# Autodesk Inventor assembly: Ambient_board_Meteostanice
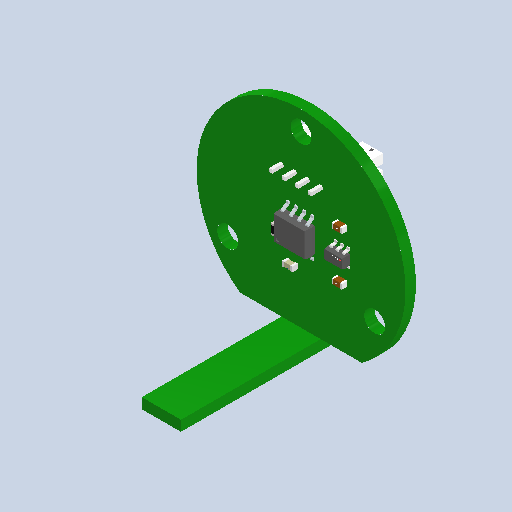
[picture p0: Inventor's stored thumbnail of the model, 512x512]
Saved by Autodesk Inventor 2025.2 (Build 292293000, 293)
## iProperties
Company: Open CASCADE
Created: 2025-02-10
Part Number: Ambient_board_Meteostanice
Description: Open CASCADE Model
Document SubType Name: Assembly
Designer: yehorderehus
Authority: Unknown
Sending System: Open CASCADE 7.5
Preprocessor: Open CASCADE STEP processor 7.5
Title: Open CASCADE Shape Model
Author: Author
## Documents named in this file (66)
- G:\.shortcut-targets-by-id\1Afqr12NmjXaFk11r_F7oLitoDl4TiMfc\Structures\assembly\Ambient_board_Meteostanice.iam
- G:\.shortcut-targets-by-id\1Afqr12NmjXaFk11r_F7oLitoDl4TiMfc\Structures\assembly\Ambient_board_Meteostanice\Ambient_board_Meteostanice\Open CASCADE STEP translator 7.5 66.ipt
- G:\.shortcut-targets-by-id\1Afqr12NmjXaFk11r_F7oLitoDl4TiMfc\Structures\assembly\Ambient_board_Meteostanice\Ambient_board_Meteostanice\Open CASCADE STEP translator 7.5 67.ipt
- G:\.shortcut-targets-by-id\1Afqr12NmjXaFk11r_F7oLitoDl4TiMfc\Structures\assembly\Ambient_board_Meteostanice\Ambient_board_Meteostanice\Open CASCADE STEP translator 7.5 68.ipt
- G:\.shortcut-targets-by-id\1Afqr12NmjXaFk11r_F7oLitoDl4TiMfc\Structures\assembly\Ambient_board_Meteostanice\Ambient_board_Meteostanice\Open CASCADE STEP translator 7.5 69.ipt
- G:\.shortcut-targets-by-id\1Afqr12NmjXaFk11r_F7oLitoDl4TiMfc\Structures\assembly\Ambient_board_Meteostanice\Ambient_board_Meteostanice\Open CASCADE STEP translator 7.5 70.ipt
- G:\.shortcut-targets-by-id\1Afqr12NmjXaFk11r_F7oLitoDl4TiMfc\Structures\assembly\Ambient_board_Meteostanice\Ambient_board_Meteostanice\Open CASCADE STEP translator 7.5 71.ipt
- G:\.shortcut-targets-by-id\1Afqr12NmjXaFk11r_F7oLitoDl4TiMfc\Structures\assembly\Ambient_board_Meteostanice\Ambient_board_Meteostanice\Open CASCADE STEP translator 7.5 72.ipt
- G:\.shortcut-targets-by-id\1Afqr12NmjXaFk11r_F7oLitoDl4TiMfc\Structures\assembly\Ambient_board_Meteostanice\Ambient_board_Meteostanice\Open CASCADE STEP translator 7.5 73.ipt
- G:\.shortcut-targets-by-id\1Afqr12NmjXaFk11r_F7oLitoDl4TiMfc\Structures\assembly\Ambient_board_Meteostanice\Ambient_board_Meteostanice\Open CASCADE STEP translator 7.5 74.ipt
- G:\.shortcut-targets-by-id\1Afqr12NmjXaFk11r_F7oLitoDl4TiMfc\Structures\assembly\Ambient_board_Meteostanice\Ambient_board_Meteostanice\Open CASCADE STEP translator 7.5 75.ipt
- G:\.shortcut-targets-by-id\1Afqr12NmjXaFk11r_F7oLitoDl4TiMfc\Structures\assembly\Ambient_board_Meteostanice\Ambient_board_Meteostanice\Open CASCADE STEP translator 7.5 76.ipt
- G:\.shortcut-targets-by-id\1Afqr12NmjXaFk11r_F7oLitoDl4TiMfc\Structures\assembly\Ambient_board_Meteostanice\Ambient_board_Meteostanice\Open CASCADE STEP translator 7.5 77.ipt
- G:\.shortcut-targets-by-id\1Afqr12NmjXaFk11r_F7oLitoDl4TiMfc\Structures\assembly\Ambient_board_Meteostanice\Ambient_board_Meteostanice\Open CASCADE STEP translator 7.5 78.ipt
- G:\.shortcut-targets-by-id\1Afqr12NmjXaFk11r_F7oLitoDl4TiMfc\Structures\assembly\Ambient_board_Meteostanice\Ambient_board_Meteostanice\Open CASCADE STEP translator 7.5 79.ipt
- G:\.shortcut-targets-by-id\1Afqr12NmjXaFk11r_F7oLitoDl4TiMfc\Structures\assembly\Ambient_board_Meteostanice\Ambient_board_Meteostanice\Open CASCADE STEP translator 7.5 80.ipt
- G:\.shortcut-targets-by-id\1Afqr12NmjXaFk11r_F7oLitoDl4TiMfc\Structures\assembly\Ambient_board_Meteostanice\Ambient_board_Meteostanice\Open CASCADE STEP translator 7.5 81.ipt
- G:\.shortcut-targets-by-id\1Afqr12NmjXaFk11r_F7oLitoDl4TiMfc\Structures\assembly\Ambient_board_Meteostanice\Ambient_board_Meteostanice\Open CASCADE STEP translator 7.5 82.ipt
- G:\.shortcut-targets-by-id\1Afqr12NmjXaFk11r_F7oLitoDl4TiMfc\Structures\assembly\Ambient_board_Meteostanice\Ambient_board_Meteostanice\Open CASCADE STEP translator 7.5 83.ipt
- G:\.shortcut-targets-by-id\1Afqr12NmjXaFk11r_F7oLitoDl4TiMfc\Structures\assembly\Ambient_board_Meteostanice\Ambient_board_Meteostanice\Open CASCADE STEP translator 7.5 84.ipt
- G:\.shortcut-targets-by-id\1Afqr12NmjXaFk11r_F7oLitoDl4TiMfc\Structures\assembly\Ambient_board_Meteostanice\Ambient_board_Meteostanice\Open CASCADE STEP translator 7.5 85.ipt
- G:\.shortcut-targets-by-id\1Afqr12NmjXaFk11r_F7oLitoDl4TiMfc\Structures\assembly\Ambient_board_Meteostanice\Ambient_board_Meteostanice\Open CASCADE STEP translator 7.5 86.ipt
- G:\.shortcut-targets-by-id\1Afqr12NmjXaFk11r_F7oLitoDl4TiMfc\Structures\assembly\Ambient_board_Meteostanice\Ambient_board_Meteostanice\Open CASCADE STEP translator 7.5 87.ipt
- G:\.shortcut-targets-by-id\1Afqr12NmjXaFk11r_F7oLitoDl4TiMfc\Structures\assembly\Ambient_board_Meteostanice\Ambient_board_Meteostanice\Open CASCADE STEP translator 7.5 88.ipt
- G:\.shortcut-targets-by-id\1Afqr12NmjXaFk11r_F7oLitoDl4TiMfc\Structures\assembly\Ambient_board_Meteostanice\Ambient_board_Meteostanice\Open CASCADE STEP translator 7.5 89.ipt
- G:\.shortcut-targets-by-id\1Afqr12NmjXaFk11r_F7oLitoDl4TiMfc\Structures\assembly\Ambient_board_Meteostanice\Ambient_board_Meteostanice\Open CASCADE STEP translator 7.5 90.ipt
- G:\.shortcut-targets-by-id\1Afqr12NmjXaFk11r_F7oLitoDl4TiMfc\Structures\assembly\Ambient_board_Meteostanice\Ambient_board_Meteostanice\Open CASCADE STEP translator 7.5 91.ipt
- G:\.shortcut-targets-by-id\1Afqr12NmjXaFk11r_F7oLitoDl4TiMfc\Structures\assembly\Ambient_board_Meteostanice\Ambient_board_Meteostanice\Open CASCADE STEP translator 7.5 92.ipt
- G:\.shortcut-targets-by-id\1Afqr12NmjXaFk11r_F7oLitoDl4TiMfc\Structures\assembly\Ambient_board_Meteostanice\Ambient_board_Meteostanice\Open CASCADE STEP translator 7.5 93.ipt
- G:\.shortcut-targets-by-id\1Afqr12NmjXaFk11r_F7oLitoDl4TiMfc\Structures\assembly\Ambient_board_Meteostanice\Ambient_board_Meteostanice\Open CASCADE STEP translator 7.5 94.ipt
- G:\.shortcut-targets-by-id\1Afqr12NmjXaFk11r_F7oLitoDl4TiMfc\Structures\assembly\Ambient_board_Meteostanice\Ambient_board_Meteostanice\Open CASCADE STEP translator 7.5 95.ipt
- G:\.shortcut-targets-by-id\1Afqr12NmjXaFk11r_F7oLitoDl4TiMfc\Structures\assembly\Ambient_board_Meteostanice\Ambient_board_Meteostanice\Open CASCADE STEP translator 7.5 96.ipt
- G:\.shortcut-targets-by-id\1Afqr12NmjXaFk11r_F7oLitoDl4TiMfc\Structures\assembly\Ambient_board_Meteostanice\Ambient_board_Meteostanice\Open CASCADE STEP translator 7.5 97.ipt
- G:\.shortcut-targets-by-id\1Afqr12NmjXaFk11r_F7oLitoDl4TiMfc\Structures\assembly\Ambient_board_Meteostanice\Ambient_board_Meteostanice\Open CASCADE STEP translator 7.5 101.ipt
- G:\.shortcut-targets-by-id\1Afqr12NmjXaFk11r_F7oLitoDl4TiMfc\Structures\assembly\Ambient_board_Meteostanice\Ambient_board_Meteostanice\Open CASCADE STEP translator 7.5 102.ipt
- G:\.shortcut-targets-by-id\1Afqr12NmjXaFk11r_F7oLitoDl4TiMfc\Structures\assembly\Ambient_board_Meteostanice\Ambient_board_Meteostanice\Open CASCADE STEP translator 7.5 103.ipt
- G:\.shortcut-targets-by-id\1Afqr12NmjXaFk11r_F7oLitoDl4TiMfc\Structures\assembly\Ambient_board_Meteostanice\Ambient_board_Meteostanice\Open CASCADE STEP translator 7.5 104.ipt
- G:\.shortcut-targets-by-id\1Afqr12NmjXaFk11r_F7oLitoDl4TiMfc\Structures\assembly\Ambient_board_Meteostanice\Ambient_board_Meteostanice\Open CASCADE STEP translator 7.5 105.ipt
- G:\.shortcut-targets-by-id\1Afqr12NmjXaFk11r_F7oLitoDl4TiMfc\Structures\assembly\Ambient_board_Meteostanice\Ambient_board_Meteostanice\Open CASCADE STEP translator 7.5 106.ipt
- G:\.shortcut-targets-by-id\1Afqr12NmjXaFk11r_F7oLitoDl4TiMfc\Structures\assembly\Ambient_board_Meteostanice\Ambient_board_Meteostanice\Open CASCADE STEP translator 7.5 107.ipt
- G:\.shortcut-targets-by-id\1Afqr12NmjXaFk11r_F7oLitoDl4TiMfc\Structures\assembly\Ambient_board_Meteostanice\Ambient_board_Meteostanice\Open CASCADE STEP translator 7.5 108.ipt
- G:\.shortcut-targets-by-id\1Afqr12NmjXaFk11r_F7oLitoDl4TiMfc\Structures\assembly\Ambient_board_Meteostanice\Ambient_board_Meteostanice\Open CASCADE STEP translator 7.5 109.ipt
- G:\.shortcut-targets-by-id\1Afqr12NmjXaFk11r_F7oLitoDl4TiMfc\Structures\assembly\Ambient_board_Meteostanice\Ambient_board_Meteostanice\Open CASCADE STEP translator 7.5 110.ipt
- G:\.shortcut-targets-by-id\1Afqr12NmjXaFk11r_F7oLitoDl4TiMfc\Structures\assembly\Ambient_board_Meteostanice\Ambient_board_Meteostanice\Open CASCADE STEP translator 7.5 111.ipt
- G:\.shortcut-targets-by-id\1Afqr12NmjXaFk11r_F7oLitoDl4TiMfc\Structures\assembly\Ambient_board_Meteostanice\Ambient_board_Meteostanice\Open CASCADE STEP translator 7.5 112.ipt
- G:\.shortcut-targets-by-id\1Afqr12NmjXaFk11r_F7oLitoDl4TiMfc\Structures\assembly\Ambient_board_Meteostanice\Ambient_board_Meteostanice\Open CASCADE STEP translator 7.5 113.ipt
- G:\.shortcut-targets-by-id\1Afqr12NmjXaFk11r_F7oLitoDl4TiMfc\Structures\assembly\Ambient_board_Meteostanice\Ambient_board_Meteostanice\Open CASCADE STEP translator 7.5 114.ipt
- G:\.shortcut-targets-by-id\1Afqr12NmjXaFk11r_F7oLitoDl4TiMfc\Structures\assembly\Ambient_board_Meteostanice\Ambient_board_Meteostanice\Open CASCADE STEP translator 7.5 115.ipt
- G:\.shortcut-targets-by-id\1Afqr12NmjXaFk11r_F7oLitoDl4TiMfc\Structures\assembly\Ambient_board_Meteostanice\Ambient_board_Meteostanice\Open CASCADE STEP translator 7.5 116.ipt
- G:\.shortcut-targets-by-id\1Afqr12NmjXaFk11r_F7oLitoDl4TiMfc\Structures\assembly\Ambient_board_Meteostanice\Ambient_board_Meteostanice\Open CASCADE STEP translator 7.5 117.ipt
- G:\.shortcut-targets-by-id\1Afqr12NmjXaFk11r_F7oLitoDl4TiMfc\Structures\assembly\Ambient_board_Meteostanice\Ambient_board_Meteostanice\Open CASCADE STEP translator 7.5 118.ipt
- G:\.shortcut-targets-by-id\1Afqr12NmjXaFk11r_F7oLitoDl4TiMfc\Structures\assembly\Ambient_board_Meteostanice\Ambient_board_Meteostanice\Open CASCADE STEP translator 7.5 119.ipt
- G:\.shortcut-targets-by-id\1Afqr12NmjXaFk11r_F7oLitoDl4TiMfc\Structures\assembly\Ambient_board_Meteostanice\Ambient_board_Meteostanice\Open CASCADE STEP translator 7.5 120.ipt
- G:\.shortcut-targets-by-id\1Afqr12NmjXaFk11r_F7oLitoDl4TiMfc\Structures\assembly\Ambient_board_Meteostanice\Ambient_board_Meteostanice\Open CASCADE STEP translator 7.5 121.ipt
- G:\.shortcut-targets-by-id\1Afqr12NmjXaFk11r_F7oLitoDl4TiMfc\Structures\assembly\Ambient_board_Meteostanice\Ambient_board_Meteostanice\Open CASCADE STEP translator 7.5 125.ipt
- G:\.shortcut-targets-by-id\1Afqr12NmjXaFk11r_F7oLitoDl4TiMfc\Structures\assembly\Ambient_board_Meteostanice\Ambient_board_Meteostanice\Open CASCADE STEP translator 7.5 126.ipt
- G:\.shortcut-targets-by-id\1Afqr12NmjXaFk11r_F7oLitoDl4TiMfc\Structures\assembly\Ambient_board_Meteostanice\Ambient_board_Meteostanice\Open CASCADE STEP translator 7.5 127.ipt
- G:\.shortcut-targets-by-id\1Afqr12NmjXaFk11r_F7oLitoDl4TiMfc\Structures\assembly\Ambient_board_Meteostanice\Ambient_board_Meteostanice\Open CASCADE STEP translator 7.5 128.ipt
- G:\.shortcut-targets-by-id\1Afqr12NmjXaFk11r_F7oLitoDl4TiMfc\Structures\assembly\Ambient_board_Meteostanice\Ambient_board_Meteostanice\Open CASCADE STEP translator 7.5 129.ipt
- G:\.shortcut-targets-by-id\1Afqr12NmjXaFk11r_F7oLitoDl4TiMfc\Structures\assembly\Ambient_board_Meteostanice\Ambient_board_Meteostanice\Open CASCADE STEP translator 7.5 130.ipt
- G:\.shortcut-targets-by-id\1Afqr12NmjXaFk11r_F7oLitoDl4TiMfc\Structures\assembly\Ambient_board_Meteostanice\Ambient_board_Meteostanice\Open CASCADE STEP translator 7.5 66_CPY1.ipt
- G:\.shortcut-targets-by-id\1Afqr12NmjXaFk11r_F7oLitoDl4TiMfc\Structures\assembly\Ambient_board_Meteostanice\Ambient_board_Meteostanice\Open CASCADE STEP translator 7.5 98_CPY.ipt
- G:\.shortcut-targets-by-id\1Afqr12NmjXaFk11r_F7oLitoDl4TiMfc\Structures\assembly\Ambient_board_Meteostanice\Ambient_board_Meteostanice\Open CASCADE STEP translator 7.5 99_CPY.ipt
- G:\.shortcut-targets-by-id\1Afqr12NmjXaFk11r_F7oLitoDl4TiMfc\Structures\assembly\Ambient_board_Meteostanice\Ambient_board_Meteostanice\Open CASCADE STEP translator 7.5 100_CPY.ipt
- G:\.shortcut-targets-by-id\1Afqr12NmjXaFk11r_F7oLitoDl4TiMfc\Structures\assembly\Ambient_board_Meteostanice\Ambient_board_Meteostanice\Open CASCADE STEP translator 7.5 123_CPY.ipt
- G:\.shortcut-targets-by-id\1Afqr12NmjXaFk11r_F7oLitoDl4TiMfc\Structures\assembly\Ambient_board_Meteostanice\Ambient_board_Meteostanice\Open CASCADE STEP translator 7.5 124_CPY.ipt
## Components (65 placed, 7 different names)
1. Open CASCADE STEP translator 7 — Rigid:1
2. Open CASCADE STEP translator 7:1
3. Open CASCADE STEP translator 7:2
4. Open CASCADE STEP translator 7:3
5. Open CASCADE STEP translator 7:4
6. Open CASCADE STEP translator 7:5
7. Open CASCADE STEP translator 7:6
8. Open CASCADE STEP translator 7:7
9. Open CASCADE STEP translator 7:8
10. Open CASCADE STEP translator 7:9
11. Open CASCADE STEP translator 7:10
12. Open CASCADE STEP translator 7:11
13. Open CASCADE STEP translator 7:12
14. Open CASCADE STEP translator 7:13
15. Open CASCADE STEP translator 7:14
16. Open CASCADE STEP translator 7:15
17. Open CASCADE STEP translator 7:16
18. Open CASCADE STEP translator 7:17
19. Open CASCADE STEP translator 7:18
20. Open CASCADE STEP translator 7:19
21. Open CASCADE STEP translator 7:20
22. Open CASCADE STEP translator 7:21
23. Open CASCADE STEP translator 7:22
24. Open CASCADE STEP translator 7:23
25. Open CASCADE STEP translator 7:24
26. Open CASCADE STEP translator 7:25
27. Open CASCADE STEP translator 7:26
28. Open CASCADE STEP translator 7:27
29. Open CASCADE STEP translator 7:28
30. Open CASCADE STEP translator 7:29
31. Open CASCADE STEP translator 7:30
32. Open CASCADE STEP translator 7:31
33. Open CASCADE STEP translator 7:35
34. Open CASCADE STEP translator 7:36
35. Open CASCADE STEP translator 7:37
36. Open CASCADE STEP translator 7:38
37. Open CASCADE STEP translator 7:39
38. Open CASCADE STEP translator 7:40
39. Open CASCADE STEP translator 7:41
40. Open CASCADE STEP translator 7:42
41. Open CASCADE STEP translator 7:43
42. Open CASCADE STEP translator 7:44
43. Open CASCADE STEP translator 7:45
44. Open CASCADE STEP translator 7:46
45. Open CASCADE STEP translator 7:47
46. Open CASCADE STEP translator 7:48
47. Open CASCADE STEP translator 7:49
48. Open CASCADE STEP translator 7:50
49. Open CASCADE STEP translator 7:51
50. Open CASCADE STEP translator 7:52
51. Open CASCADE STEP translator 7:53
52. Open CASCADE STEP translator 7:54
53. Open CASCADE STEP translator 7:55
54. Open CASCADE STEP translator 7:59
55. Open CASCADE STEP translator 7:60
56. Open CASCADE STEP translator 7:61
57. Open CASCADE STEP translator 7:62
58. Open CASCADE STEP translator 7:63
59. Open CASCADE STEP translator 7:64
60. Open CASCADE STEP translator 7.5 66_CPY1:1 — Flush:1, Flush:2, Flush:3, Flush:4, Flush:5, Flush:6, Flush:7, Flush:8, Flush:9, Flush:10, Flush:11, Flush:12, Flush:13, Mate:1, Flush:14, Rigid:1
61. Open CASCADE STEP translator 7.5 98_CPY:1 — Flush:3, Flush:8, Flush:13
62. Open CASCADE STEP translator 7.5 99_CPY:1 — Flush:5, Flush:10, Mate:1
63. Open CASCADE STEP translator 7.5 100_CPY:1 — Flush:4, Flush:9, Flush:14
64. Open CASCADE STEP translator 7.5 123_CPY:1 — Flush:1, Flush:7, Flush:11
65. Open CASCADE STEP translator 7.5 124_CPY:1 — Flush:2, Flush:6, Flush:12
## Relationships (16: Flush 14, Mate 1, WeldJoint 1)
- Flush:1 (-0.82 mm): Open CASCADE STEP translator 7.5 66_CPY1:1 ↔ Open CASCADE STEP translator 7.5 123_CPY:1
- Flush:2 (-0.87 mm): Open CASCADE STEP translator 7.5 66_CPY1:1 ↔ Open CASCADE STEP translator 7.5 124_CPY:1
- Flush:3 (-1.45 mm): Open CASCADE STEP translator 7.5 66_CPY1:1 ↔ Open CASCADE STEP translator 7.5 98_CPY:1
- Flush:4 (-0.766 mm): Open CASCADE STEP translator 7.5 66_CPY1:1 ↔ Open CASCADE STEP translator 7.5 100_CPY:1
- Flush:5 (-0.766 mm): Open CASCADE STEP translator 7.5 66_CPY1:1 ↔ Open CASCADE STEP translator 7.5 99_CPY:1
- Flush:6 (2.962 mm): Open CASCADE STEP translator 7.5 66_CPY1:1 ↔ Open CASCADE STEP translator 7.5 124_CPY:1
- Flush:7 (6.09 mm): Open CASCADE STEP translator 7.5 66_CPY1:1 ↔ Open CASCADE STEP translator 7.5 123_CPY:1
- Flush:8 (1.54 mm): Open CASCADE STEP translator 7.5 66_CPY1:1 ↔ Open CASCADE STEP translator 7.5 98_CPY:1
- Flush:9 (2.8 mm): Open CASCADE STEP translator 7.5 66_CPY1:1 ↔ Open CASCADE STEP translator 7.5 100_CPY:1
- Flush:10 (1.85 mm): Open CASCADE STEP translator 7.5 66_CPY1:1 ↔ Open CASCADE STEP translator 7.5 99_CPY:1
- Flush:11 (3.312 mm): Open CASCADE STEP translator 7.5 66_CPY1:1 ↔ Open CASCADE STEP translator 7.5 123_CPY:1
- Flush:12 (6.04 mm): Open CASCADE STEP translator 7.5 66_CPY1:1 ↔ Open CASCADE STEP translator 7.5 124_CPY:1
- Flush:13 (1.83 mm): Open CASCADE STEP translator 7.5 66_CPY1:1 ↔ Open CASCADE STEP translator 7.5 98_CPY:1
- Mate:1 (-4.03 mm): Open CASCADE STEP translator 7.5 66_CPY1:1 ↔ Open CASCADE STEP translator 7.5 99_CPY:1
- Flush:14 (1.23 mm): Open CASCADE STEP translator 7.5 66_CPY1:1 ↔ Open CASCADE STEP translator 7.5 100_CPY:1
- Rigid:1 [WeldJoint]: Open CASCADE STEP translator 7 ↔ Open CASCADE STEP translator 7.5 66_CPY1:1
